# Autodesk Inventor assembly: frame
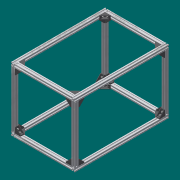
[picture p0: Inventor's stored thumbnail of the model, 180x180]
Saved by Autodesk Inventor 2016 SP1 (Build 200210100, 210)
## iProperties
Created: 2016-02-10
Part Number: frame
Document SubType Name: Assembly
Designer: Sawaiz
Author: Sawaiz
## Documents named in this file (4)
- C:\Users\sawai\OneDrive\projects\modularRICHFrame\frame\frame.iam
- C:\Users\sawai\OneDrive\projects\modularRICHFrame\frame\face.iam
- C:\Users\sawai\OneDrive\projects\modularRICHFrame\frame\hfs5-2020Depth.ipt
- C:\Users\sawai\OneDrive\projects\modularRICHFrame\hardware\angleBracket.iam
## Components (22 placed, 3 different names)
1. face:1 [sub-assembly] — Flush:1, Flush:2, Symmetry:1, Symmetry:2, Symmetry:3, Flush:3, Flush:4, Flush:5, Flush:6, Mate:2, Mate:3, Flush:7, Flush:8, Flush:9, Flush:10, Flush:11, Flush:12, Flush:13, Flush:14, Flush:39, Mate:22, Mate:25, Flush:70, Mate:36, Mate:40, Mate:43, Mate:49, Mate:53
2. face:2 [sub-assembly] — Flush:1, Flush:2, Symmetry:1, Symmetry:2, Symmetry:3, Mate:1, Flush:15, Mate:23, Mate:26, Mate:37, Mate:38, Flush:72, Flush:74, Mate:44, Mate:47, Flush:83, Mate:48, Mate:51
3. hfs5-2020Depth:1 — Mate:1, Flush:3, Flush:12, Flush:13, Flush:14, Mate:35, Mate:42, Mate:45
4. hfs5-2020Depth:2 — Flush:4, Flush:9, Flush:10, Flush:11, Flush:15, Mate:27, Mate:41, Mate:46
5. hfs5-2020Depth:3 — Flush:6, Mate:2, Mate:3, Mate:39, Mate:52
6. hfs5-2020Depth:4 — Flush:5, Flush:7, Flush:8, Flush:38, Mate:24, Mate:50
7. angleBracket:9 [sub-assembly] — Flush:37, Flush:38, Flush:41, Mate:26, Mate:27
8. angleBracket:10 [sub-assembly] — Flush:36, Flush:37, Mate:22, Flush:40, Mate:24
9. angleBracket:11 [sub-assembly] — Flush:35, Flush:36, Flush:39, Mate:23, Flush:40
10. angleBracket:12 [sub-assembly] — Flush:35, Flush:41, Mate:25
11. angleBracket:13 [sub-assembly] — Flush:65, Flush:66, Flush:67, Flush:68, Mate:37
12. angleBracket:14 [sub-assembly] — Flush:63, Flush:64, Flush:68, Flush:69, Mate:39
13. angleBracket:15 [sub-assembly] — Flush:63, Flush:69, Mate:38
14. angleBracket:16 [sub-assembly] — Flush:64, Flush:65, Flush:66, Mate:35, Flush:67, Flush:70, Mate:36
15. angleBracket:17 [sub-assembly] — Flush:71, Mate:42, Mate:43
16. angleBracket:18 [sub-assembly] — Flush:71, Flush:72, Mate:44, Mate:45
17. angleBracket:19 [sub-assembly] — Flush:73, Mate:40, Mate:41
18. angleBracket:20 [sub-assembly] — Flush:73, Flush:74, Mate:46, Mate:47
19. angleBracket:21 [sub-assembly] — Flush:78, Flush:79, Flush:80, Mate:53
20. angleBracket:22 [sub-assembly] — Flush:79, Flush:80, Flush:81, Mate:51, Mate:52
21. angleBracket:23 [sub-assembly] — Flush:77, Flush:78, Flush:82, Mate:49, Mate:50
22. angleBracket:24 [sub-assembly] — Flush:77, Flush:81, Flush:82, Flush:83, Mate:48
## Relationships (79: Flush 48, Mate 28, Symmetry 3)
- Flush:1: face:1 ↔ face:2
- Flush:2: face:1 ↔ face:2
- Symmetry:1: face:1 ↔ face:2
- Symmetry:2: face:1 ↔ face:2
- Symmetry:3: face:1 ↔ face:2
- Mate:1: face:2 ↔ hfs5-2020Depth:1
- Flush:3: face:1 ↔ hfs5-2020Depth:1
- Flush:4: face:1 ↔ hfs5-2020Depth:2
- Flush:5: face:1 ↔ hfs5-2020Depth:4
- Flush:6: face:1 ↔ hfs5-2020Depth:3
- Mate:2: face:1 ↔ hfs5-2020Depth:3
- Mate:3: face:1 ↔ hfs5-2020Depth:3
- Flush:7: face:1 ↔ hfs5-2020Depth:4
- Flush:8: face:1 ↔ hfs5-2020Depth:4
- Flush:9: face:1 ↔ hfs5-2020Depth:2
- Flush:10: face:1 ↔ hfs5-2020Depth:2
- Flush:11: face:1 ↔ hfs5-2020Depth:2
- Flush:12: face:1 ↔ hfs5-2020Depth:1
- Flush:13: face:1 ↔ hfs5-2020Depth:1
- Flush:14: face:1 ↔ hfs5-2020Depth:1
- Flush:15: face:2 ↔ hfs5-2020Depth:2
- Flush:35: angleBracket:11 ↔ angleBracket:12
- Flush:36: angleBracket:10 ↔ angleBracket:11
- Flush:37: angleBracket:9 ↔ angleBracket:10
- Flush:38: hfs5-2020Depth:4 ↔ angleBracket:9
- Flush:39: face:1 ↔ angleBracket:11
- Mate:22: face:1 ↔ angleBracket:10
- Mate:23: face:2 ↔ angleBracket:11
- Flush:40: angleBracket:10 ↔ angleBracket:11
- Mate:24: hfs5-2020Depth:4 ↔ angleBracket:10
- Flush:41: angleBracket:9 ↔ angleBracket:12
- Mate:25: face:1 ↔ angleBracket:12
- Mate:26: face:2 ↔ angleBracket:9
- Mate:27: hfs5-2020Depth:2 ↔ angleBracket:9
- [Flush]: angleBracket:15 ↔ angleBracket:16
- [Flush]: angleBracket:14 ↔ angleBracket:15
- [Flush]: angleBracket:13 ↔ angleBracket:14
- [Flush]: angleBracket:14 ↔ angleBracket:15
- [Flush]: angleBracket:13 ↔ angleBracket:16
- Flush:63: angleBracket:14 ↔ angleBracket:15
- Flush:64: angleBracket:14 ↔ angleBracket:16
- Flush:65: angleBracket:13 ↔ angleBracket:16
- Flush:66: angleBracket:13 ↔ angleBracket:16
- Mate:35: hfs5-2020Depth:1 ↔ angleBracket:16
- Flush:67: angleBracket:13 ↔ angleBracket:16
- Flush:68: angleBracket:13 ↔ angleBracket:14
- Flush:69: angleBracket:14 ↔ angleBracket:15
- Flush:70: face:1 ↔ angleBracket:16
- Mate:36: face:1 ↔ angleBracket:16
- Mate:37: face:2 ↔ angleBracket:13
- Mate:38: face:2 ↔ angleBracket:15
- Mate:39: hfs5-2020Depth:3 ↔ angleBracket:14
- Flush:71: angleBracket:17 ↔ angleBracket:18
- Flush:72: face:2 ↔ angleBracket:18
- Flush:73: angleBracket:19 ↔ angleBracket:20
- Flush:74: face:2 ↔ angleBracket:20
- Mate:40: face:1 ↔ angleBracket:19
- Mate:41: hfs5-2020Depth:2 ↔ angleBracket:19
- Mate:42: hfs5-2020Depth:1 ↔ angleBracket:17
- Mate:43: face:1 ↔ angleBracket:17
- Mate:44: face:2 ↔ angleBracket:18
- Mate:45: hfs5-2020Depth:1 ↔ angleBracket:18
- Mate:46: hfs5-2020Depth:2 ↔ angleBracket:20
- Mate:47: face:2 ↔ angleBracket:20
- [Flush]: angleBracket:21 ↔ angleBracket:22
- [Flush]: angleBracket:23 ↔ angleBracket:24
- Flush:77: angleBracket:23 ↔ angleBracket:24
- Flush:78: angleBracket:21 ↔ angleBracket:23
- Flush:79: angleBracket:21 ↔ angleBracket:22
- Flush:80: angleBracket:21 ↔ angleBracket:22
- Flush:81: angleBracket:22 ↔ angleBracket:24
- Flush:82: angleBracket:23 ↔ angleBracket:24
- Flush:83: face:2 ↔ angleBracket:24
- Mate:48: face:2 ↔ angleBracket:24
- Mate:49: face:1 ↔ angleBracket:23
- Mate:50: hfs5-2020Depth:4 ↔ angleBracket:23
- Mate:51: face:2 ↔ angleBracket:22
- Mate:52: hfs5-2020Depth:3 ↔ angleBracket:22
- Mate:53: face:1 ↔ angleBracket:21
## Named parameters: d109_d55 = 0 mm, d110_d56 = 0 mm, d111_d57 = 0 mm, d112_d62 = 0 mm, d113_d64 = 0 mm, d147_d135 = 0 mm, d148_d137 = 0 mm
